# Autodesk Inventor assembly: stepper
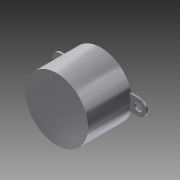
[picture p0: Inventor's stored thumbnail of the model, 180x180]
Saved by Autodesk Inventor 2014 (Build 180170000, 170)
## iProperties
Created: 2015-01-06
Part Number: stepper
Document SubType Name: Assembly
Designer: cruiser
Author: cruiser
## Documents named in this file (3)
- C:\Users\cruiser\Desktop\models\3d printers\laserresin2\stepper.iam
- C:\Users\cruiser\Desktop\models\3d printers\laserresin2\small_stepper.ipt
- C:\Users\cruiser\Desktop\models\3d printers\laserresin2\small_stepper_shaft.ipt
## Components (2 placed, 2 different names)
1. small_stepper:1 — Mate:1, Rotational:1
2. small_stepper_shaft:1 — Mate:1, Rotational:1
## Relationships (2: Mate 1, RevoluteJoint 1)
- Mate:1: small_stepper:1 ↔ small_stepper_shaft:1
- Rotational:1 [RevoluteJoint]: small_stepper:1 ↔ small_stepper_shaft:1
